# Autodesk Inventor assembly: gripper
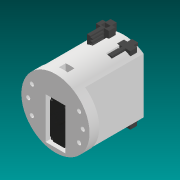
[picture p0: Inventor's stored thumbnail of the model, 180x180]
Saved by Autodesk Inventor 2020.3 (Build 243373000, 373)
## iProperties
Created: 2020-05-25
Part Number: gripper
Document SubType Name: Assembly
Designer: Svend
Author: Svend
## Documents named in this file (5)
- C:\Users\Svend\OneDrive\Documents\GitHub\BeerMinder\3D-model\gripper\gripper.iam
- C:\Users\Svend\OneDrive\Documents\GitHub\BeerMinder\3D-model\gripper\slider.ipt
- C:\Users\Svend\OneDrive\Documents\GitHub\BeerMinder\3D-model\gripper\grippershape.ipt
- C:\Users\Svend\OneDrive\Documents\GitHub\BeerMinder\3D-model\servo\MG_996R.iam
- C:\Users\Svend\OneDrive\Documents\GitHub\BeerMinder\3D-model\pulleys\Gear 16×1-0.1-V1.1.ipt
## Components (5 placed, 4 different names)
1. slider:1 — Angle:1, Flush:1, Mate:1, Mate:6, Mate:7, Angle:2
2. slider:2 — Angle:1, Flush:1, Mate:1
3. grippershape:1 — Mate:5, Mate:6, Mate:7, Mate:8
4. MG_996R:1 [sub-assembly] — Mate:4, Angle:2, Mate:9
5. Gear 16×1-0.1-V1.1:1 — Mate:4, Mate:5, Mate:8, Mate:9
## Relationships (10: Mate 7, Angle 2, Flush 1)
- Angle:1 (0 deg): slider:1 ↔ slider:2
- Flush:1: slider:1 ↔ slider:2
- Mate:1 (15.45 mm): slider:1 ↔ slider:2
- Mate:4: MG_996R:1 ↔ Gear 16×1-0.1-V1.1:1
- Mate:5: grippershape:1 ↔ Gear 16×1-0.1-V1.1:1
- Mate:6 (0.05 mm): slider:1 ↔ grippershape:1
- Mate:7 (0.05 mm): slider:1 ↔ grippershape:1
- Mate:8 (0.1 mm): grippershape:1 ↔ Gear 16×1-0.1-V1.1:1
- Angle:2 (180 deg): slider:1 ↔ MG_996R:1
- Mate:9: MG_996R:1 ↔ Gear 16×1-0.1-V1.1:1
